# Autodesk Inventor assembly: 000-hand-grab-v4
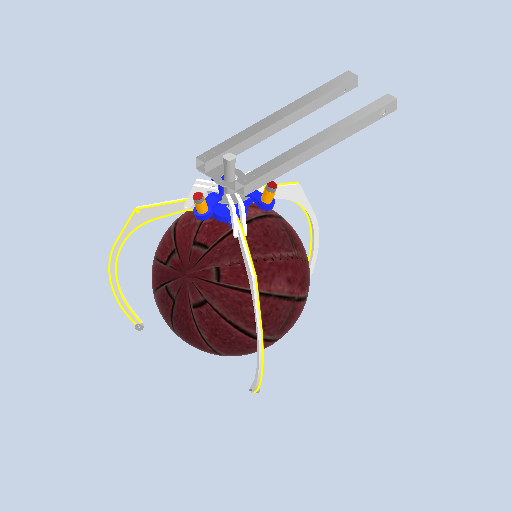
[picture p0: Inventor's stored thumbnail of the model, 512x512]
Saved by Autodesk Inventor 2025.2 (Build 292293000, 293)
## iProperties
Created: 2024-10-07
Part Number: 000-hand-grab-v4
Document SubType Name: Assembly
Designer: haruy
Author: haruy
## Documents named in this file (16)
- C:\Users\haruy\Documents\ロボコン\NHK2025\cad\nagahisa\hand\grab\000-hand-grab-v4.iam
- C:\Users\haruy\Documents\ロボコン\NHK2025\cad\nagahisa\hand\grab\hand-grab-v1-MDF-air-Base.ipt
- C:\Users\haruy\Documents\ロボコン\NHK2025\cad\nagahisa\hand\grab\hand-grab-v1-POM-link-F-1.ipt
- C:\Users\haruy\Documents\ロボコン\NHK2025\cad\nagahisa\hand\grab\hand-grab-v1-3DP-link-F-2.ipt
- C:\Users\haruy\Documents\ロボコン\NHK2025\cad\nagahisa\hand\grab\bearing-10-3.ipt
- C:\Users\haruy\Documents\ロボコン\NHK2025\cad\nagahisa\hand\grab\C-SEFL683ZZ.ipt
- C:\Users\haruy\Documents\ロボコン\NHK2025\cad\nagahisa\hand\grab\E-NTBGT13-8.iam
- C:\Users\haruy\Documents\ロボコン\NHK2025\cad\basket-ball.ipt
- C:\Users\haruy\Documents\ロボコン\NHK2025\cad\000_parts\エアシリンダー\airclinder\CDJ2B16-15Z-B(0_1_0).iam
- C:\Users\haruy\Documents\ロボコン\NHK2025\cad\nagahisa\hand\grab\hand-grab-v1-ASP-arm-support.ipt
- C:\Users\haruy\Documents\ロボコン\NHK2025\cad\nagahisa\hand\grab\hand-grab-v1-MDF-arm.ipt
- C:\Users\haruy\Documents\ロボコン\NHK2025\cad\nagahisa\hand\grab\hand-grab-v3-3DP-light_F.ipt
- C:\Users\haruy\Documents\ロボコン\NHK2025\cad\000_parts\センサー\E18_D80NK.ipt
- C:\Users\haruy\Documents\ロボコン\NHK2025\cad\nagahisa\hand\grab\hand-grab-v3-3DP-spesa_1.ipt
- C:\Users\haruy\Documents\ロボコン\NHK2025\cad\nagahisa\hand\grab\hand-grab-v3-Plate-ASP_F.ipt
- C:\Users\haruy\Documents\ロボコン\NHK2025\cad\nagahisa\hand\grab\hand-grab-v4-ASP_1.ipt
## Components (42 placed, 15 different names)
1. hand-grab-v1-MDF-air-Base:1 — 挿入:2, 挿入:3, 挿入:4, 挿入:5, 挿入:6, 挿入:7, 挿入:8, 挿入:9, 挿入:10, 挿入:11, 挿入:12, 挿入:13, 挿入:30, 挿入:38, 挿入:39, 挿入:40, 挿入:41, 挿入:42, 挿入:43, 挿入:47, 挿入:48, 挿入:49
2. hand-grab-v1-POM-link-F-1:1 — 挿入:2, 挿入:3
3. hand-grab-v1-POM-link-F-1:2 — 挿入:4, 挿入:5
4. hand-grab-v1-POM-link-F-1:3 — 挿入:6, 挿入:7
5. hand-grab-v1-POM-link-F-1:4 — 挿入:8, 挿入:9
6. hand-grab-v1-POM-link-F-1:5 — 挿入:10, 挿入:11
7. hand-grab-v1-POM-link-F-1:6 — 挿入:12, 挿入:13, 角度:1, 挿入:29
8. hand-grab-v1-3DP-link-F-2:1 — 挿入:16, 挿入:18, 挿入:20, 角度:1, 挿入:31
9. bearing-10-3:1 — 挿入:15, 正接:7
10. bearing-10-3:2 — 挿入:15, 挿入:16
11. bearing-10-3:3
12. bearing-10-3:4 — 挿入:18
13. bearing-10-3:5 — 挿入:20
14. bearing-10-3:6
15. basket-ball:1 — 正接:6
16. CDJ2B16-15Z-B(0_1_0):1 [sub-assembly] — 挿入:30, 挿入:31
17. hand-grab-v1-ASP-arm-support:1
18. hand-grab-v1-ASP-arm-support:2
19. hand-grab-v3-3DP-light_F:1 — 挿入:38, 挿入:39, 挿入:44
20. hand-grab-v3-3DP-light_F:2 — 挿入:40, 挿入:41, 挿入:46
21. hand-grab-v3-3DP-light_F:3 — 挿入:42, 挿入:43, 挿入:45
22. E18_D80NK:1 — 挿入:44
23. E18_D80NK:2 — 挿入:46
24. E18_D80NK:3 — 挿入:45
25. hand-grab-v3-3DP-spesa_1:1 — 挿入:48, 挿入:50
26. hand-grab-v3-3DP-spesa_1:2 — 挿入:47
27. hand-grab-v3-3DP-spesa_1:3 — 挿入:49, 挿入:51
28. hand-grab-v3-Plate-ASP_F:1 — 挿入:50, 挿入:51, 挿入:52, 挿入:53, 挿入:54, 挿入:55
29. hand-grab-v4-ASP_1:1 — 挿入:52, 挿入:53
30. hand-grab-v4-ASP_1:2 — 挿入:54, 挿入:55
31. hand-grab-v1-MDF-arm:1 — 挿入:36, 挿入:37, 正接:7
32. E-NTBGT13-8:1 [sub-assembly] — 正接:6, 挿入:36
33. C-SEFL683ZZ:1 — 挿入:29, 挿入:37
34. C-SEFL683ZZ:2
35. hand-grab-v1-MDF-arm:2
36. E-NTBGT13-8:2 [sub-assembly]
37. C-SEFL683ZZ:3
38. C-SEFL683ZZ:4
39. hand-grab-v1-MDF-arm:3
40. E-NTBGT13-8:3 [sub-assembly]
41. C-SEFL683ZZ:5
42. C-SEFL683ZZ:6
## Component patterns: (3 elements, first: hand-grab-v1-MDF-arm:1 + E-NTBGT13-8:1 + C-SEFL683ZZ:1 + C-SEFL683ZZ:2)
## Relationships (44: Insert 41, Tangent 2, Angle 1)
- 挿入:2 [Insert]: hand-grab-v1-MDF-air-Base:1 ↔ hand-grab-v1-POM-link-F-1:1
- 挿入:3 [Insert]: hand-grab-v1-MDF-air-Base:1 ↔ hand-grab-v1-POM-link-F-1:1
- 挿入:4 [Insert]: hand-grab-v1-MDF-air-Base:1 ↔ hand-grab-v1-POM-link-F-1:2
- 挿入:5 [Insert]: hand-grab-v1-MDF-air-Base:1 ↔ hand-grab-v1-POM-link-F-1:2
- 挿入:6 [Insert]: hand-grab-v1-MDF-air-Base:1 ↔ hand-grab-v1-POM-link-F-1:3
- 挿入:7 [Insert]: hand-grab-v1-MDF-air-Base:1 ↔ hand-grab-v1-POM-link-F-1:3
- 挿入:8 [Insert]: hand-grab-v1-MDF-air-Base:1 ↔ hand-grab-v1-POM-link-F-1:4
- 挿入:9 [Insert]: hand-grab-v1-MDF-air-Base:1 ↔ hand-grab-v1-POM-link-F-1:4
- 挿入:10 [Insert]: hand-grab-v1-MDF-air-Base:1 ↔ hand-grab-v1-POM-link-F-1:5
- 挿入:11 [Insert]: hand-grab-v1-MDF-air-Base:1 ↔ hand-grab-v1-POM-link-F-1:5
- 挿入:12 [Insert]: hand-grab-v1-MDF-air-Base:1 ↔ hand-grab-v1-POM-link-F-1:6
- 挿入:13 [Insert]: hand-grab-v1-MDF-air-Base:1 ↔ hand-grab-v1-POM-link-F-1:6
- 挿入:15 [Insert]: bearing-10-3:1 ↔ bearing-10-3:2
- 挿入:16 [Insert] (0.25 mm): hand-grab-v1-3DP-link-F-2:1 ↔ bearing-10-3:2
- [Insert]: bearing-10-3:3 ↔ bearing-10-3:4
- 挿入:18 [Insert] (0.25 mm): hand-grab-v1-3DP-link-F-2:1 ↔ bearing-10-3:4
- [Insert]: bearing-10-3:5 ↔ bearing-10-3:6
- 挿入:20 [Insert] (0.25 mm): hand-grab-v1-3DP-link-F-2:1 ↔ bearing-10-3:5
- 角度:1 [Angle] (0 deg): hand-grab-v1-POM-link-F-1:6 ↔ hand-grab-v1-3DP-link-F-2:1
- 挿入:29 [Insert] (0.2 mm): hand-grab-v1-POM-link-F-1:6 ↔ C-SEFL683ZZ:1
- 挿入:30 [Insert]: hand-grab-v1-MDF-air-Base:1 ↔ CDJ2B16-15Z-B(0_1_0):1
- 正接:6 [Tangent]: basket-ball:1 ↔ E-NTBGT13-8:1
- 挿入:31 [Insert] (4 mm): hand-grab-v1-3DP-link-F-2:1 ↔ CDJ2B16-15Z-B(0_1_0):1
- 挿入:36 [Insert]: hand-grab-v1-MDF-arm:1 ↔ E-NTBGT13-8:1
- 挿入:37 [Insert]: hand-grab-v1-MDF-arm:1 ↔ C-SEFL683ZZ:1
- 正接:7 [Tangent]: bearing-10-3:1 ↔ hand-grab-v1-MDF-arm:1
- 挿入:38 [Insert]: hand-grab-v1-MDF-air-Base:1 ↔ hand-grab-v3-3DP-light_F:1
- 挿入:39 [Insert]: hand-grab-v1-MDF-air-Base:1 ↔ hand-grab-v3-3DP-light_F:1
- 挿入:40 [Insert]: hand-grab-v1-MDF-air-Base:1 ↔ hand-grab-v3-3DP-light_F:2
- 挿入:41 [Insert]: hand-grab-v1-MDF-air-Base:1 ↔ hand-grab-v3-3DP-light_F:2
- 挿入:42 [Insert]: hand-grab-v1-MDF-air-Base:1 ↔ hand-grab-v3-3DP-light_F:3
- 挿入:43 [Insert]: hand-grab-v1-MDF-air-Base:1 ↔ hand-grab-v3-3DP-light_F:3
- 挿入:44 [Insert]: hand-grab-v3-3DP-light_F:1 ↔ E18_D80NK:1
- 挿入:45 [Insert]: hand-grab-v3-3DP-light_F:3 ↔ E18_D80NK:3
- 挿入:46 [Insert]: hand-grab-v3-3DP-light_F:2 ↔ E18_D80NK:2
- 挿入:47 [Insert]: hand-grab-v1-MDF-air-Base:1 ↔ hand-grab-v3-3DP-spesa_1:2
- 挿入:48 [Insert]: hand-grab-v1-MDF-air-Base:1 ↔ hand-grab-v3-3DP-spesa_1:1
- 挿入:49 [Insert]: hand-grab-v1-MDF-air-Base:1 ↔ hand-grab-v3-3DP-spesa_1:3
- 挿入:50 [Insert]: hand-grab-v3-3DP-spesa_1:1 ↔ hand-grab-v3-Plate-ASP_F:1
- 挿入:51 [Insert]: hand-grab-v3-3DP-spesa_1:3 ↔ hand-grab-v3-Plate-ASP_F:1
- 挿入:52 [Insert]: hand-grab-v3-Plate-ASP_F:1 ↔ hand-grab-v4-ASP_1:1
- 挿入:53 [Insert]: hand-grab-v3-Plate-ASP_F:1 ↔ hand-grab-v4-ASP_1:1
- 挿入:54 [Insert]: hand-grab-v3-Plate-ASP_F:1 ↔ hand-grab-v4-ASP_1:2
- 挿入:55 [Insert]: hand-grab-v3-Plate-ASP_F:1 ↔ hand-grab-v4-ASP_1:2
## Named parameters: d16_d14 = 0 mm, d18_d14 = 0 mm
